# Autodesk Inventor assembly: bepf_kolo
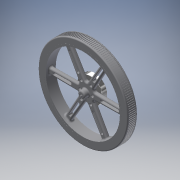
[picture p0: Inventor's stored thumbnail of the model, 180x180]
Saved by Autodesk Inventor 2017 (Build 210142000, 142)
## iProperties
Part Number: bepf_kolo
Material: Ogólny
Document SubType Name: Assembly
Designer: gagato
Author: gagato
## Documents named in this file (4)
- C:\Users\gagato\Documents\bepf\bepf_kolo.iam
- C:\Users\gagato\Documents\bepf\bepf_kolo_felga.ipt
- C:\Users\gagato\Documents\bepf\bepf_kolo_opona.ipt
- C:\Users\gagato\Documents\bepf\bepf_kolo_adapter_walu_fi6.ipt
## Components (3 placed, 3 different names)
1. bepf_kolo_felga:1 — Zestawiający:1, Zestawiający:2, Równoległy:1, Obrót:1, Zestawiający:3, Zestawiający:4, Zestawiający:5
2. bepf_kolo_opona:1 — Zestawiający:2, Równoległy:1, Obrót:1
3. bepf_kolo_adapter_walu_fi6:1 — Zestawiający:3, Zestawiający:4, Zestawiający:5
## Relationships (7: Mate 5, Flush 1, RelateRotation 1)
- Zestawiający:1 [Mate]: bepf_kolo_felga:1
- Zestawiający:2 [Mate]: bepf_kolo_felga:1 ↔ bepf_kolo_opona:1
- Równoległy:1 [Flush]: bepf_kolo_felga:1 ↔ bepf_kolo_opona:1
- Obrót:1 [RelateRotation] (1 ul): bepf_kolo_felga:1 ↔ bepf_kolo_opona:1
- Zestawiający:3 [Mate]: bepf_kolo_felga:1 ↔ bepf_kolo_adapter_walu_fi6:1
- Zestawiający:4 [Mate]: bepf_kolo_felga:1 ↔ bepf_kolo_adapter_walu_fi6:1
- Zestawiający:5 [Mate]: bepf_kolo_felga:1 ↔ bepf_kolo_adapter_walu_fi6:1
